# Autodesk Inventor assembly: Auto Arm
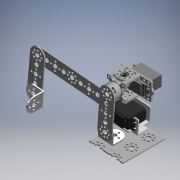
[picture p0: Inventor's stored thumbnail of the model, 180x180]
Saved by Autodesk Inventor 2019 (Build 230136000, 136)
## iProperties
Part Number: Auto Arm
Document SubType Name: Assembly
Designer: Delta
Author: Delta
## Documents named in this file (9)
- C:\Robotics\2019-20_CAD\Collection\Auto Arm.iam
- C:\Robotics\COTSParts\Tetrix\Pitsco Education-739273.ipt
- C:\Robotics\COTSParts\Tetrix\39060_txm-standard servo bracket.ipt
- C:\Robotics\COTSParts\Tetrix\39274_txm-flat64mmx27mm.ipt
- C:\Robotics\COTSParts\Tetrix\39197_txm-485hb standard servo with horn.ipt
- C:\Robotics\COTSParts\Tetrix\Servo with servo blocks.ipt
- C:\Robotics\COTSParts\Tetrix\Tetrix Flat bar 160 mm.ipt
- C:\Robotics\COTSParts\Tetrix\Tetrix bracket - angle.ipt
- C:\Robotics\2019-20_CAD\Collection\auto arm plate.ipt
## Components (10 placed, 8 different names)
1. Pitsco Education-739273:1 — Mate:10, Mate:11, Mate:12, Mate:16, Mate:17, Mate:18
2. 39060_txm-standard servo bracket:1 — Mate:1, Mate:2, Angle:1, Mate:24, Mate:26, Mate:28, Angle:4
3. 39274_txm-flat64mmx27mm:1 — Mate:3, Mate:4, Mate:7, Mate:8, Mate:9
4. 39197_txm-485hb standard servo with horn:1 — Mate:1, Mate:2, Angle:1, Mate:3, Mate:4
5. Pitsco Education-739273:2 — Mate:5, Mate:6, Mate:21, Mate:22, Mate:23, Angle:3
6. Servo with servo blocks:1 — Mate:5, Mate:6
7. Tetrix Flat bar 160 mm:1 — Mate:7, Mate:8, Mate:9, Mate:10, Mate:11, Mate:12
8. Tetrix bracket - angle:1 — Mate:16, Mate:17, Mate:18
9. Tetrix bracket - angle:2 — Mate:21, Mate:22, Mate:23, Angle:3, Mate:25, Mate:27, Angle:5
10. auto arm plate:1 — Mate:24, Mate:25, Mate:26, Mate:27, Mate:28, Angle:4, Angle:5
## Relationships (27: Mate 23, Angle 4)
- Mate:1: 39060_txm-standard servo bracket:1 ↔ 39197_txm-485hb standard servo with horn:1
- Mate:2: 39060_txm-standard servo bracket:1 ↔ 39197_txm-485hb standard servo with horn:1
- Angle:1 (0 deg): 39060_txm-standard servo bracket:1 ↔ 39197_txm-485hb standard servo with horn:1
- Mate:3: 39274_txm-flat64mmx27mm:1 ↔ 39197_txm-485hb standard servo with horn:1
- Mate:4: 39274_txm-flat64mmx27mm:1 ↔ 39197_txm-485hb standard servo with horn:1
- Mate:5: Pitsco Education-739273:2 ↔ Servo with servo blocks:1
- Mate:6: Pitsco Education-739273:2 ↔ Servo with servo blocks:1
- Mate:7: 39274_txm-flat64mmx27mm:1 ↔ Tetrix Flat bar 160 mm:1
- Mate:8: 39274_txm-flat64mmx27mm:1 ↔ Tetrix Flat bar 160 mm:1
- Mate:9: 39274_txm-flat64mmx27mm:1 ↔ Tetrix Flat bar 160 mm:1
- Mate:10: Pitsco Education-739273:1 ↔ Tetrix Flat bar 160 mm:1
- Mate:11: Pitsco Education-739273:1 ↔ Tetrix Flat bar 160 mm:1
- Mate:12: Pitsco Education-739273:1 ↔ Tetrix Flat bar 160 mm:1
- Mate:16: Pitsco Education-739273:1 ↔ Tetrix bracket - angle:1
- Mate:17: Pitsco Education-739273:1 ↔ Tetrix bracket - angle:1
- Mate:18: Pitsco Education-739273:1 ↔ Tetrix bracket - angle:1
- Mate:21: Pitsco Education-739273:2 ↔ Tetrix bracket - angle:2
- Mate:22: Pitsco Education-739273:2 ↔ Tetrix bracket - angle:2
- Mate:23: Pitsco Education-739273:2 ↔ Tetrix bracket - angle:2
- Angle:3 (0 deg): Pitsco Education-739273:2 ↔ Tetrix bracket - angle:2
- Mate:24: 39060_txm-standard servo bracket:1 ↔ auto arm plate:1
- Mate:25: Tetrix bracket - angle:2 ↔ auto arm plate:1
- Mate:26: 39060_txm-standard servo bracket:1 ↔ auto arm plate:1
- Mate:27: Tetrix bracket - angle:2 ↔ auto arm plate:1
- Mate:28: 39060_txm-standard servo bracket:1 ↔ auto arm plate:1
- Angle:4 (0 deg): 39060_txm-standard servo bracket:1 ↔ auto arm plate:1
- Angle:5 (0 deg): Tetrix bracket - angle:2 ↔ auto arm plate:1
